# Autodesk Inventor assembly: ASY PNS 1750 filter-distribution-system 1200
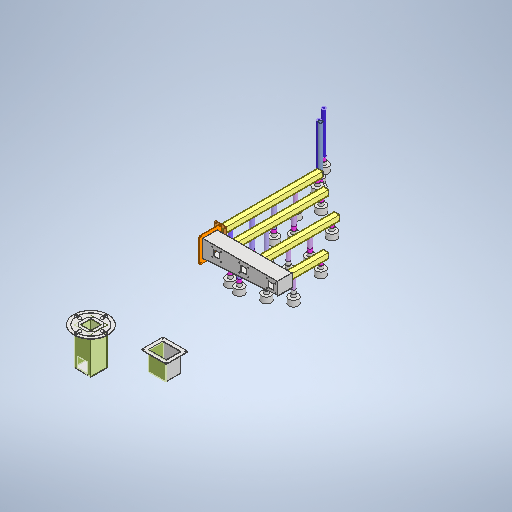
[picture p0: Inventor's stored thumbnail of the model, 512x512]
Saved by Autodesk Inventor 2025 (Build 290162010, 162A)
## iProperties
Created: 2025-06-24
Part Number: ASY PNS 1750 filter-distribution-system 1200
Document SubType Name: Assembly
Designer: user
Author: user
## Documents named in this file (11)
- C:\Users\pokla\Documents\Inventor\ANP--Antipayuta\ASY PNS 1750 filter-distribution-system 1200.iam
- C:\Users\pokla\Documents\Inventor\ANP--Antipayuta\Workspaces\Workspace\filter-distribution-system\PNS 1759 DIM filter-distribution-system 1200.ipt
- C:\Users\pokla\Documents\Inventor\ANP--Antipayuta\Workspaces\Workspace\filter-distribution-system\PNS 754 FDS 1200 FLANGE.ipt
- C:\Users\pokla\Documents\Inventor\ANP--Antipayuta\Workspaces\Workspace\filter-distribution-system\PNS 752 FDS 1200 FLANGE 2.ipt
- C:\Users\pokla\Documents\Inventor\ANP--Antipayuta\PNS 765 FDS 1200 CUP 1.ipt
- C:\Users\pokla\Documents\Inventor\ANP--Antipayuta\PNS 1757 FDS 1200x50 FLANGE.ipt
- C:\Users\pokla\Documents\Inventor\ANP--Antipayuta\PNS 1762 FDS 1200x50 column.ipt
- C:\Users\pokla\Documents\Inventor\ANP--Antipayuta\FDS 1400\ASY ANP 1490 FDS one way.iam
- C:\Users\pokla\Documents\Inventor\ANP--Antipayuta\FDS 1400\ASY ANP 1424 FDS way 4.iam
- C:\Users\pokla\Documents\Inventor\ANP--Antipayuta\Workspaces\Workspace\filter-distribution-system\PNS 753 FDS 1200 FLANGE 2.ipt
- C:\Users\pokla\Documents\Inventor\ANP--Antipayuta\FDS 1400\ANP 1421 FDS Diam way flange 1.ipt
## Components (12 placed, 10 different names)
1. PNS 751 DIM filter-distribution-system 1200.ipt:1 — Mate:4, Mate:5
2. PNS 754 FDS 1200 FLANGE.ipt:1 — Mate:1, Flush:1, Flush:2
3. PNS 752 FDS 1200 FLANGE 2.ipt:1 — Rigid:1, Flush:1, Mate:6, Flush:3, Flush:4
4. PNS 752 FDS 1200 FLANGE 2.ipt:2 — Rigid:1, Mate:1, Flush:2
5. PNS 765 FDS 1200 CUP 1.ipt:1 — Mate:6, Flush:3, Flush:4
6. PNS 1757 FDS 1200x50 FLANGE:1 — Rigid:35, Flush:5, Mate:7, Flush:6
7. PNS 1762 FDS 1200x50 column:1 — Rigid:35
8. ASY ANP 1424 FDS way 4.iam:1 [sub-assembly]
9. ASY ANP 1490 FDS one way:1 [sub-assembly]
10. PNS 753 FDS 1200 FLANGE 2:1 — Rigid:36, Rigid:37
11. PNS 753 FDS 1200 FLANGE 2:2 — Rigid:36
12. ANP 1421 FDS Diam way flange 1:1 — Rigid:37
## Relationships (15: Flush 6, Mate 5, WeldJoint 4)
- Rigid:1 [WeldJoint]: PNS 752 FDS 1200 FLANGE 2.ipt:1 ↔ PNS 752 FDS 1200 FLANGE 2.ipt:2
- Mate:1: PNS 754 FDS 1200 FLANGE.ipt:1 ↔ PNS 752 FDS 1200 FLANGE 2.ipt:2
- Flush:1: PNS 754 FDS 1200 FLANGE.ipt:1 ↔ PNS 752 FDS 1200 FLANGE 2.ipt:1
- Flush:2: PNS 754 FDS 1200 FLANGE.ipt:1 ↔ PNS 752 FDS 1200 FLANGE 2.ipt:2
- Mate:4: PNS 751 DIM filter-distribution-system 1200.ipt:1
- Mate:5: PNS 751 DIM filter-distribution-system 1200.ipt:1
- Mate:6: PNS 752 FDS 1200 FLANGE 2.ipt:1 ↔ PNS 765 FDS 1200 CUP 1.ipt:1
- Flush:3: PNS 752 FDS 1200 FLANGE 2.ipt:1 ↔ PNS 765 FDS 1200 CUP 1.ipt:1
- Flush:4: PNS 752 FDS 1200 FLANGE 2.ipt:1 ↔ PNS 765 FDS 1200 CUP 1.ipt:1
- Rigid:35 [WeldJoint]: PNS 1757 FDS 1200x50 FLANGE:1 ↔ PNS 1762 FDS 1200x50 column:1
- Flush:5: PNS 1757 FDS 1200x50 FLANGE:1
- Mate:7: PNS 1757 FDS 1200x50 FLANGE:1
- Flush:6: PNS 1757 FDS 1200x50 FLANGE:1
- Rigid:36 [WeldJoint]: PNS 753 FDS 1200 FLANGE 2:1 ↔ PNS 753 FDS 1200 FLANGE 2:2
- Rigid:37 [WeldJoint]: PNS 753 FDS 1200 FLANGE 2:1 ↔ ANP 1421 FDS Diam way flange 1:1
